# Autodesk Inventor assembly: am-3322+RhinoTrackDriveModule
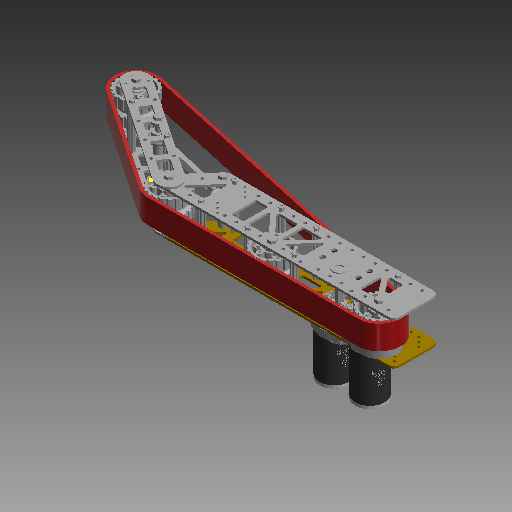
[picture p0: Inventor's stored thumbnail of the model, 512x512]
Saved by Autodesk Inventor 2017.2 (Build 212233000, 233)
## iProperties
Created: 2015-12-17
Part Number: am-3322+RhinoTrackDriveModule
Description: STEP AP203
Document SubType Name: Assembly
Designer: steele
Mass: 4285.93 g
Surface Area: 10743.9 cm^2
Volume: 2788.38 cm^3
Density: 1.53707 g/cm^3
Sending System: SolidWorks 2014
Preprocessor: SwSTEP 2.0
Title: am-3322 Rhino Track Drive Module.STEP
Revision Number: ANY
## Documents named in this file (29)
- D:\snobotics\CAD-Development\robSteele\SnoBotics2016\RhinoTrackDriveModule\am-3322+RhinoTrackDriveModule.iam
- D:\snobotics\CAD-Development\robSteele\SnoBotics2016\RhinoTrackDriveModule\am-3319 Inside Plate.ipt
- D:\snobotics\CAD-Development\robSteele\SnoBotics2016\RhinoTrackDriveModule\20T pulley back to back.iam
- D:\snobotics\CAD-Development\robSteele\SnoBotics2016\RhinoTrackDriveModule\am-1393 375 washer.ipt
- D:\snobotics\CAD-Development\robSteele\SnoBotics2016\RhinoTrackDriveModule\am-3320 Upper Bar.ipt
- D:\snobotics\CAD-Development\robSteele\SnoBotics2016\RhinoTrackDriveModule\Track Belt.ipt
- D:\snobotics\CAD-Development\robSteele\SnoBotics2016\RhinoTrackDriveModule\am-2598_107 2016 KOP Toughbox Mini.iam
- D:\snobotics\CAD-Development\robSteele\SnoBotics2016\RhinoTrackDriveModule\am-3318 Outside Plate.ipt
- D:\snobotics\CAD-Development\robSteele\SnoBotics2016\RhinoTrackDriveModule\FR8ZZ Hex Bearing.ipt
- D:\snobotics\CAD-Development\robSteele\SnoBotics2016\RhinoTrackDriveModule\am-0207a 250 Sprocket and Pulley Spacer.ipt
- D:\snobotics\CAD-Development\robSteele\SnoBotics2016\RhinoTrackDriveModule\10-24 Hex Washer Rolling x 1.25_93882A213.ipt
- D:\snobotics\CAD-Development\robSteele\SnoBotics2016\RhinoTrackDriveModule\425-5M-15.ipt
- D:\snobotics\CAD-Development\robSteele\SnoBotics2016\RhinoTrackDriveModule\500EX Hex Hub.ipt
- D:\snobotics\CAD-Development\robSteele\SnoBotics2016\RhinoTrackDriveModule\BHCS 10-32 x 1000_SBHCSCREW 0.19-32x0.5-HX-C.ipt
- D:\snobotics\CAD-Development\robSteele\SnoBotics2016\RhinoTrackDriveModule\10-32 Nylock Nut.ipt
- D:\snobotics\CAD-Development\robSteele\SnoBotics2016\RhinoTrackDriveModule\0985x0420 PVC Spacer.ipt
- D:\snobotics\CAD-Development\robSteele\SnoBotics2016\RhinoTrackDriveModule\Churro 3375.ipt
- D:\snobotics\CAD-Development\robSteele\SnoBotics2016\RhinoTrackDriveModule\FHTS 0.25-20-0.75_FHTS 0.25-20-G-0.75-C.ipt
- D:\snobotics\CAD-Development\robSteele\SnoBotics2016\RhinoTrackDriveModule\375-16 x 4.25 Hex Bolt_HFBOLT 0.375-16x2.5x1-C.ipt
- D:\snobotics\CAD-Development\robSteele\SnoBotics2016\RhinoTrackDriveModule\3-8-16 NyLock Nut - Mcm 95615A140_95615A140.ipt
- D:\snobotics\CAD-Development\robSteele\SnoBotics2016\RhinoTrackDriveModule\10-32x0625_shcs_HX-SHCS 0.19-32x1.375x1-C.ipt
- D:\snobotics\CAD-Development\robSteele\SnoBotics2016\RhinoTrackDriveModule\187x385 spacer 13RS038518.ipt
- D:\snobotics\CAD-Development\robSteele\SnoBotics2016\RhinoTrackDriveModule\am-0243 spacer 1860x0420.ipt
- D:\snobotics\CAD-Development\robSteele\SnoBotics2016\RhinoTrackDriveModule\500 Hex Collar Clamp.iam
- D:\snobotics\CAD-Development\robSteele\SnoBotics2016\RhinoTrackDriveModule\Spacer am-1181.ipt
- D:\snobotics\CAD-Development\robSteele\SnoBotics2016\RhinoTrackDriveModule\Round Collar 375.ipt
- D:\snobotics\CAD-Development\robSteele\SnoBotics2016\RhinoTrackDriveModule\am-2243 brass spacer.ipt
- D:\snobotics\CAD-Development\robSteele\SnoBotics2016\RhinoTrackDriveModule\am-3321 turnbuckle.iam
- D:\snobotics\autodesk\2016\FRC KOP 2016\Motors\MOT_CIM-Motor_217-2000.iam
## Components (92 placed, 91 different names)
1. am-3319 Inside Plate_1
2. 20T pulley back to back_2 [sub-assembly]
3. am-1393 375 washer_3
4. am-3320 Upper Bar_4
5. am-3320 Upper Bar_5
6. 20T pulley back to back_6 [sub-assembly]
7. Track Belt_7
8. am-2598_107 2016 KOP Toughbox Mini_8 [sub-assembly] — Insert:1, Insert:2
9. am-3318 Outside Plate_9
10. 20T pulley back to back_10 [sub-assembly]
11. 20T pulley back to back_11 [sub-assembly]
12. FR8ZZ Hex Bearing_12
13. am-0207a 250 Sprocket and Pulley Spacer_13
14. 10-24 Hex Washer Rolling x 1.25_93882A213_14
15. 10-24 Hex Washer Rolling x 1.25_93882A213_15
16. 10-24 Hex Washer Rolling x 1.25_93882A213_16
17. 425-5M-15_17
18. 500EX Hex Hub_18
19. BHCS 10-32 x 1000_SBHCSCREW 0.19-32x0.5-HX-C_19
20. BHCS 10-32 x 1000_SBHCSCREW 0.19-32x0.5-HX-C_20
21. BHCS 10-32 x 1000_SBHCSCREW 0.19-32x0.5-HX-C_21
22. BHCS 10-32 x 1000_SBHCSCREW 0.19-32x0.5-HX-C_22
23. BHCS 10-32 x 1000_SBHCSCREW 0.19-32x0.5-HX-C_23
24. BHCS 10-32 x 1000_SBHCSCREW 0.19-32x0.5-HX-C_24
25. 10-32 Nylock Nut_25
26. 10-32 Nylock Nut_26
27. 10-32 Nylock Nut_27
28. 10-32 Nylock Nut_28
29. 10-32 Nylock Nut_29
30. 10-32 Nylock Nut_30
31. am-1393 375 washer_31
32. am-1393 375 washer_32
33. 0985x0420 PVC Spacer_33
34. 0985x0420 PVC Spacer_34
35. Churro 3375_35
36. Churro 3375_36
37. Churro 3375_37
38. Churro 3375_38
39. Churro 3375_39
40. Churro 3375_40
41. Churro 3375_41
42. FHTS 0.25-20-0.75_FHTS 0.25-20-G-0.75-C_42
43. FHTS 0.25-20-0.75_FHTS 0.25-20-G-0.75-C_43
44. FHTS 0.25-20-0.75_FHTS 0.25-20-G-0.75-C_44
45. FHTS 0.25-20-0.75_FHTS 0.25-20-G-0.75-C_45
46. FHTS 0.25-20-0.75_FHTS 0.25-20-G-0.75-C_46
47. FHTS 0.25-20-0.75_FHTS 0.25-20-G-0.75-C_47
48. FHTS 0.25-20-0.75_FHTS 0.25-20-G-0.75-C_48
49. FHTS 0.25-20-0.75_FHTS 0.25-20-G-0.75-C_49
50. FHTS 0.25-20-0.75_FHTS 0.25-20-G-0.75-C_50
51. FHTS 0.25-20-0.75_FHTS 0.25-20-G-0.75-C_51
52. FHTS 0.25-20-0.75_FHTS 0.25-20-G-0.75-C_52
53. FHTS 0.25-20-0.75_FHTS 0.25-20-G-0.75-C_53
54. FHTS 0.25-20-0.75_FHTS 0.25-20-G-0.75-C_54
55. FHTS 0.25-20-0.75_FHTS 0.25-20-G-0.75-C_55
56. 375-16 x 4.25 Hex Bolt_HFBOLT 0.375-16x2.5x1-C_56
57. 375-16 x 4.25 Hex Bolt_HFBOLT 0.375-16x2.5x1-C_57
58. 375-16 x 4.25 Hex Bolt_HFBOLT 0.375-16x2.5x1-C_58
59. 3-8-16 NyLock Nut - Mcm 95615A140_95615A140_59
60. 3-8-16 NyLock Nut - Mcm 95615A140_95615A140_60
61. 3-8-16 NyLock Nut - Mcm 95615A140_95615A140_61
62. 10-32x0625_shcs_HX-SHCS 0.19-32x1.375x1-C_62
63. 10-32x0625_shcs_HX-SHCS 0.19-32x1.375x1-C_63
64. 10-32x0625_shcs_HX-SHCS 0.19-32x1.375x1-C_64
65. 10-32x0625_shcs_HX-SHCS 0.19-32x1.375x1-C_65
66. FHTS 0.25-20-0.75_FHTS 0.25-20-G-0.75-C_66
67. FHTS 0.25-20-0.75_FHTS 0.25-20-G-0.75-C_67
68. FHTS 0.25-20-0.75_FHTS 0.25-20-G-0.75-C_68
69. FHTS 0.25-20-0.75_FHTS 0.25-20-G-0.75-C_69
70. am-1393 375 washer_70
71. 187x385 spacer 13RS038518_71
72. 375-16 x 4.25 Hex Bolt_HFBOLT 0.375-16x2.5x1-C_72
73. 3-8-16 NyLock Nut - Mcm 95615A140_95615A140_73
74. 3-8-16 NyLock Nut - Mcm 95615A140_95615A140_74
75. 375-16 x 4.25 Hex Bolt_HFBOLT 0.375-16x2.5x1-C_75
76. am-0243 spacer 1860x0420_76
77. am-0243 spacer 1860x0420_77
78. 500 Hex Collar Clamp_78 [sub-assembly]
79. Churro 3375_79
80. Churro 3375_80
81. 375-16 x 4.25 Hex Bolt_HFBOLT 0.375-16x2.5x1-C_81
82. 3-8-16 NyLock Nut - Mcm 95615A140_95615A140_82
83. Spacer am-1181_83
84. Round Collar 375_84
85. Round Collar 375_85
86. am-2243 brass spacer_86
87. am-2243 brass spacer_87
88. am-1393 375 washer_88
89. am-1393 375 washer_89
90. am-3321 turnbuckle_90 [sub-assembly]
91. MOT_CIM-Motor_217-2000:1 [sub-assembly] — Insert:1
92. MOT_CIM-Motor_217-2000:2 [sub-assembly] — Insert:2
## Relationships (2: Insert 2)
- Insert:1: am-2598_107 2016 KOP Toughbox Mini_8 ↔ MOT_CIM-Motor_217-2000:1
- Insert:2: am-2598_107 2016 KOP Toughbox Mini_8 ↔ MOT_CIM-Motor_217-2000:2
